# Autodesk Inventor assembly: bot
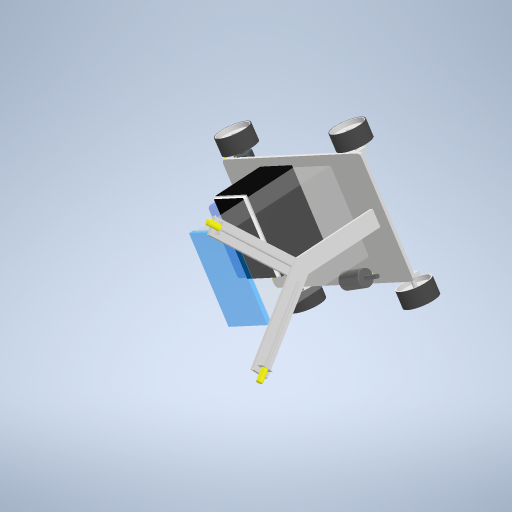
[picture p0: Inventor's stored thumbnail of the model, 512x512]
Saved by Autodesk Inventor 2023 (Build 270158000, 158)
## iProperties
Created: 2022-08-22
Part Number: bot
Document SubType Name: Assembly
Designer: Sachin
Author: Sachin
## Documents named in this file (9)
- C:\Users\Disha Hondadkatti\Downloads\Telegram Desktop\bot.iam
- C:\Users\Disha Hondadkatti\Downloads\Telegram Desktop\base.ipt
- C:\Users\Disha Hondadkatti\Downloads\Telegram Desktop\WHEEL 2.ipt
- C:\Users\Disha Hondadkatti\Downloads\Telegram Desktop\DC MOTOR.ipt
- C:\Users\Disha Hondadkatti\Downloads\Telegram Desktop\box.ipt
- C:\Users\Disha Hondadkatti\Downloads\Telegram Desktop\battery.ipt
- C:\Users\Disha Hondadkatti\Downloads\Telegram Desktop\jar.ipt
- C:\Users\Disha Hondadkatti\Downloads\Telegram Desktop\spray.ipt
- C:\Users\Disha Hondadkatti\Downloads\Telegram Desktop\stand.ipt
## Components (14 placed, 8 different names)
1. base:1 — Mate:1, Mate:2, Mate:3, Mate:4, Mate:5, Mate:6, Mate:7, Mate:12, Mate:13, Mate:14, Mate:16, Mate:18, Mate:19, Mate:20, Mate:21
2. WHEEL 2:1 — Mate:1, Mate:3
3. WHEEL 2:2 — Mate:2, Mate:4
4. DC MOTOR:1 — Mate:5, Mate:6, Mate:9, Mate:10
5. DC MOTOR:2 — Mate:7, Mate:8, Mate:11
6. WHEEL 2:3 — Mate:8, Mate:11
7. WHEEL 2:4 — Mate:9, Mate:10
8. box:1 — Mate:12, Mate:13, Mate:15
9. battery:1 — Mate:14, Mate:15, Mate:17
10. jar:1 — Mate:16, Mate:17
11. DC MOTOR:3 — Mate:18
12. spray:1 — Mate:22, Mate:23, Mate:25
13. stand:1 — Mate:19, Mate:20, Mate:21, Mate:22, Mate:23, Mate:24
14. spray:2 — Mate:24, Mate:25
## Relationships (25: Mate 25)
- Mate:1: base:1 ↔ WHEEL 2:1
- Mate:2: base:1 ↔ WHEEL 2:2
- Mate:3: base:1 ↔ WHEEL 2:1
- Mate:4: base:1 ↔ WHEEL 2:2
- Mate:5: base:1 ↔ DC MOTOR:1
- Mate:6: base:1 ↔ DC MOTOR:1
- Mate:7: base:1 ↔ DC MOTOR:2
- Mate:8: DC MOTOR:2 ↔ WHEEL 2:3
- Mate:9: DC MOTOR:1 ↔ WHEEL 2:4
- Mate:10: DC MOTOR:1 ↔ WHEEL 2:4
- Mate:11: DC MOTOR:2 ↔ WHEEL 2:3
- Mate:12: base:1 ↔ box:1
- Mate:13: base:1 ↔ box:1
- Mate:14: base:1 ↔ battery:1
- Mate:15: box:1 ↔ battery:1
- Mate:16: base:1 ↔ jar:1
- Mate:17: battery:1 ↔ jar:1
- Mate:18: base:1 ↔ DC MOTOR:3
- Mate:19: base:1 ↔ stand:1
- Mate:20: base:1 ↔ stand:1
- Mate:21: base:1 ↔ stand:1
- Mate:22: spray:1 ↔ stand:1
- Mate:23: spray:1 ↔ stand:1
- Mate:24: stand:1 ↔ spray:2
- Mate:25: spray:1 ↔ spray:2
